# Autodesk Inventor assembly: VersaPlanetary_v1_Single_Stage_10_1_with_BAG
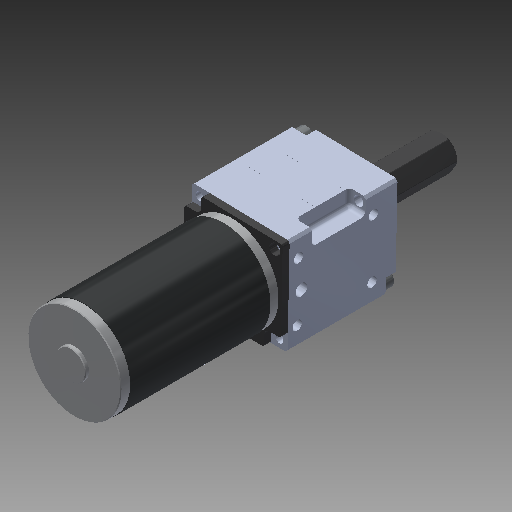
[picture p0: Inventor's stored thumbnail of the model, 512x512]
Saved by Autodesk Inventor 2019 (Build 230136000, 136)
## iProperties
Created: 2015-01-07
Part Number: VersaPlanetary_v1_Single_Stage_10_1_with_BAG
Description: STEP AP214
Document SubType Name: Assembly
Designer: josh
Mass: 158.31 g
Surface Area: 575.499 cm^2
Volume: 158.31 cm^3
Density: 1 g/cm^3
Sending System: SolidWorks 2014
Preprocessor: SwSTEP 2.0
Title: VersaPlanetary 1-Stage with BAG Motor.STEP
Revision Number: ANY
## Documents named in this file (10)
- D:\Synthesis Robots\Epsilon\Epsilon Grabbers\Bag Motor parts\VersaPlanetary_v1_Single_Stage_10_1_with_BAG.iam
- D:\Synthesis Robots\Epsilon\Epsilon Grabbers\Bag Motor parts\217-2742-001 Rev4.ipt
- D:\Synthesis Robots\Epsilon\Epsilon Grabbers\Bag Motor parts\217-2625-002 Rev1.ipt
- D:\Synthesis Robots\Epsilon\Epsilon Grabbers\Bag Motor parts\217-2625-018 Rev1_98541A410.ipt
- D:\Synthesis Robots\Epsilon\Epsilon Grabbers\Bag Motor parts\Ouput Shafts^VersaPlanetary_500 Hex.iam
- D:\Synthesis Robots\Epsilon\Epsilon Grabbers\Bag Motor parts\217-3564-000 Rev1_BAG.iam
- D:\Synthesis Robots\Epsilon\Epsilon Grabbers\Bag Motor parts\Input Housing^VersaPlanetary.iam
- D:\Synthesis Robots\Epsilon\Epsilon Grabbers\Bag Motor parts\217-2816 Rev1.iam
- D:\Synthesis Robots\Epsilon\Epsilon Grabbers\Bag Motor parts\SSA_SSA0832-1250ZC.ipt
- D:\Synthesis Robots\Epsilon\Epsilon Grabbers\Bag Motor parts\VersaPlanetary_7_1_Gear_Kit_217-3102 (1).iam
## Components (11 placed, 11 different names)
1. 217-2742-001 Rev4_1 — Mate:14, Flush:2, Mate:20, Mate:21
2. 217-2742-001 Rev4_2 — Mate:18, Flush:1
3. 217-2625-002 Rev1_3 — Mate:2, Mate:3, Mate:9, Mate:10, Mate:11, Mate:12, Mate:13, Mate:14, Mate:18, Flush:1, Flush:2, Mate:19
4. 217-2625-018 Rev1_98541A410_4 — Mate:19
5. Ouput Shafts^VersaPlanetary_500 Hex_6 [sub-assembly] — Mate:20, Mate:21
6. 217-3564-000 Rev1_BAG_7 [sub-assembly] — Mate:1, Mate:15, Mate:16, Mate:17
7. Input Housing^VersaPlanetary_8 [sub-assembly] — Mate:1, Mate:6, Mate:7, Mate:8, Mate:15, Mate:16, Mate:17
8. 217-2816 Rev1_9 [sub-assembly] — Mate:4, Mate:5, Mate:6, Mate:13
9. SSA_SSA0832-1250ZC_11 — Mate:5, Mate:7, Mate:9, Mate:12
10. SSA_SSA0832-1250ZC_12 — Mate:4, Mate:8, Mate:10, Mate:11
11. VersaPlanetary_7_1_Gear_Kit_217-3102 (1):1 [sub-assembly] — Mate:2, Mate:3
## Relationships (23: Mate 21, Flush 2)
- Mate:1: 217-3564-000 Rev1_BAG_7 ↔ Input Housing^VersaPlanetary_8
- Mate:2: 217-2625-002 Rev1_3 ↔ VersaPlanetary_7_1_Gear_Kit_217-3102 (1):1
- Mate:3: 217-2625-002 Rev1_3 ↔ VersaPlanetary_7_1_Gear_Kit_217-3102 (1):1
- Mate:4: 217-2816 Rev1_9 ↔ SSA_SSA0832-1250ZC_12
- Mate:5: 217-2816 Rev1_9 ↔ SSA_SSA0832-1250ZC_11
- Mate:6: Input Housing^VersaPlanetary_8 ↔ 217-2816 Rev1_9
- Mate:7: Input Housing^VersaPlanetary_8 ↔ SSA_SSA0832-1250ZC_11
- Mate:8: Input Housing^VersaPlanetary_8 ↔ SSA_SSA0832-1250ZC_12
- Mate:9: 217-2625-002 Rev1_3 ↔ SSA_SSA0832-1250ZC_11
- Mate:10: 217-2625-002 Rev1_3 ↔ SSA_SSA0832-1250ZC_12
- Mate:11: 217-2625-002 Rev1_3 ↔ SSA_SSA0832-1250ZC_12
- Mate:12: 217-2625-002 Rev1_3 ↔ SSA_SSA0832-1250ZC_11
- Mate:13: 217-2625-002 Rev1_3 ↔ 217-2816 Rev1_9
- Mate:14: 217-2742-001 Rev4_1 ↔ 217-2625-002 Rev1_3
- Mate:15: 217-3564-000 Rev1_BAG_7 ↔ Input Housing^VersaPlanetary_8
- Mate:16: 217-3564-000 Rev1_BAG_7 ↔ Input Housing^VersaPlanetary_8
- Mate:17: 217-3564-000 Rev1_BAG_7 ↔ Input Housing^VersaPlanetary_8
- Mate:18: 217-2742-001 Rev4_2 ↔ 217-2625-002 Rev1_3
- Flush:1: 217-2742-001 Rev4_2 ↔ 217-2625-002 Rev1_3
- Flush:2: 217-2742-001 Rev4_1 ↔ 217-2625-002 Rev1_3
- Mate:19: 217-2625-002 Rev1_3 ↔ 217-2625-018 Rev1_98541A410_4
- Mate:20: 217-2742-001 Rev4_1 ↔ Ouput Shafts^VersaPlanetary_500 Hex_6
- Mate:21: 217-2742-001 Rev4_1 ↔ Ouput Shafts^VersaPlanetary_500 Hex_6
